# Autodesk Inventor assembly: CABEZAL
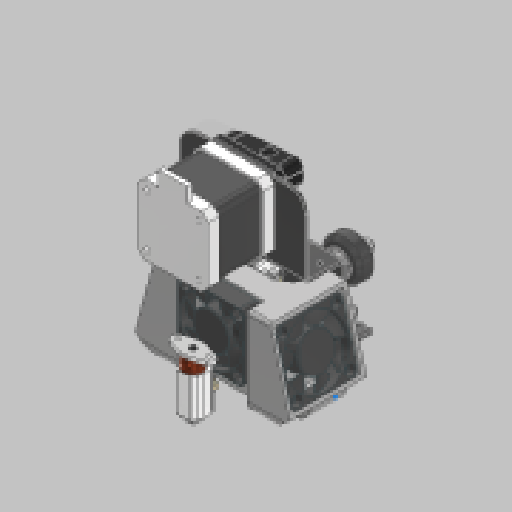
[picture p0: Inventor's stored thumbnail of the model, 512x512]
Saved by Autodesk Inventor 2025.3 (Build 293356000, 356)
## iProperties
Created: 2025-10-28
Part Number: CABEZAL
Document SubType Name: Assembly
Designer: Inema
Author: Inema
## Documents named in this file (6)
- C:\Users\Inema\OneDrive - INEMA S.A\Escritorio\Modelo Ender 3\CABEZAL.iam
- C:\Users\Inema\OneDrive - INEMA S.A\Escritorio\Modelo Ender 3\ASM Extruder.iam
- C:\Users\Inema\OneDrive - INEMA S.A\Escritorio\Modelo Ender 3\ASM Printing Head.iam
- C:\Users\Inema\OneDrive - INEMA S.A\Escritorio\Modelo Ender 3\mS_Ender_Dual_4010_1.1\mS_Ender_Dual_4010_1.1\mS_Ender_Dual_4010_1.1.ipt
- C:\Users\Inema\OneDrive - INEMA S.A\Escritorio\Modelo Ender 3\Nozzle fan.ipt
- C:\Users\Inema\OneDrive - INEMA S.A\Escritorio\Modelo Ender 3\3d-touch-v30.ipt
## Components (7 placed, 6 different names)
1. ASM Extruder_162 [sub-assembly]
2. ASM Printing Head_167 [sub-assembly] — Insertar:1, Coincidencia:2
3. mS_Ender_Dual_4010_1.1:1 — Insertar:1, Coincidencia:2
4. Nozzle fan_172
5. Nozzle fan:2
6. Nozzle fan:3
7. 3d-touch-v30:1
## Relationships (5: Mate 2, Angle 1, Flush 1, Insert 1)
- [Mate]: ASM Extruder_162 ↔ ASM Printing Head_167
- [Angle] (180 deg): ASM Extruder_162 ↔ ASM Printing Head_167
- [Flush] (-1.45 mm): ASM Extruder_162 ↔ ASM Printing Head_167
- Insertar:1: ASM Printing Head_167 ↔ mS_Ender_Dual_4010_1.1:1
- Coincidencia:2 [Mate]: ASM Printing Head_167 ↔ mS_Ender_Dual_4010_1.1:1
